# Autodesk Inventor assembly: wormGear
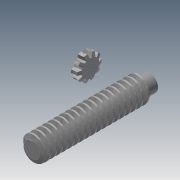
[picture p0: Inventor's stored thumbnail of the model, 180x180]
Saved by Autodesk Inventor 2018 (Build 220112000, 112)
## iProperties
Created: 2020-02-25
Part Number: wormGear
Document SubType Name: Assembly
Designer: anirudh
Author: anirudh
## Documents named in this file (3)
- D:\Silicon Sharks\2019-2020\servoBox\wormGear.iam
- D:\Silicon Sharks\2019-2020\servoBox\servoGear.ipt
- D:\Silicon Sharks\2019-2020\servoBox\wormGear\Design Accelerator\Worm Gears1.iam
## Components (2 placed, 2 different names)
1. servoGear:1 — Mate:1
2. Worm Gears:1 [sub-assembly] — Mate:1
## Relationships (1: Mate 1)
- Mate:1: servoGear:1 ↔ Worm Gears:1
